# Autodesk Inventor assembly: Ensamble JTDM
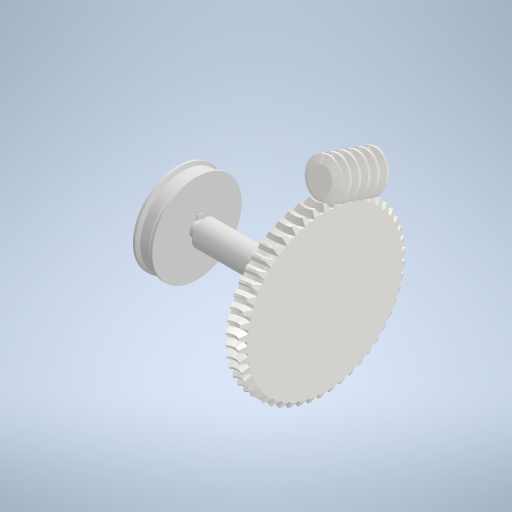
[picture p0: Inventor's stored thumbnail of the model, 512x512]
Saved by Autodesk Inventor 2024 (Build 280153000, 153)
## iProperties
Created: 2024-03-14
Part Number: Ensamble JTDM
Document SubType Name: Assembly
Designer: jtdia
Author: jtdia
## Documents named in this file (6)
- C:\Users\jtdia\OneDrive\Documentos\5to Semestre 2024\Dinámica Lab\Ensamble JTDM.iam
- C:\Users\jtdia\OneDrive\Documentos\5to Semestre 2024\Dinámica Lab\Piezas de esambleje\POLEA.ipt
- C:\Users\jtdia\OneDrive\Documentos\5to Semestre 2024\Dinámica Lab\Piezas de esambleje\ENGRANE.ipt
- C:\Users\jtdia\OneDrive\Documentos\5to Semestre 2024\Dinámica Lab\Piezas de esambleje\EJE_CUÑEROS.ipt
- C:\Users\jtdia\OneDrive\Documentos\5to Semestre 2024\Dinámica Lab\Piezas de esambleje\CUÑA.ipt
- C:\Users\jtdia\OneDrive\Documentos\5to Semestre 2024\Dinámica Lab\Ensamble JTDM\Design Accelerator\Worm Gears1.iam
## Components (6 placed, 5 different names)
1. POLEA:1 — Cylindrical:1, Flush:1, Mate:2
2. ENGRANE:1 — Rotational:1, Mate:1
3. EJE_CUÑEROS:1 — Cylindrical:1, Flush:1, Rotational:1, Mate:1, Rigid:1, Mate:2, Rigid:2, Rotational:2
4. CUÑA:1 — Rigid:1
5. CUÑA:2 — Rigid:2
6. Worm Gears:1 [sub-assembly] — Rotational:2
## Relationships (8: RevoluteJoint 2, Mate 2, WeldJoint 2, CylindricalJoint 1, Flush 1)
- Cylindrical:1: POLEA:1 ↔ EJE_CUÑEROS:1
- Flush:1: POLEA:1 ↔ EJE_CUÑEROS:1
- Rotational:1 [RevoluteJoint]: ENGRANE:1 ↔ EJE_CUÑEROS:1
- Mate:1: ENGRANE:1 ↔ EJE_CUÑEROS:1
- Rigid:1 [WeldJoint]: EJE_CUÑEROS:1 ↔ CUÑA:1
- Mate:2: POLEA:1 ↔ EJE_CUÑEROS:1
- Rigid:2 [WeldJoint]: EJE_CUÑEROS:1 ↔ CUÑA:2
- Rotational:2 [RevoluteJoint]: EJE_CUÑEROS:1 ↔ Worm Gears:1
